# Autodesk Inventor assembly: power
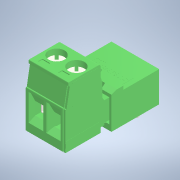
[picture p0: Inventor's stored thumbnail of the model, 180x180]
Saved by Autodesk Inventor 2021 (Build 250183000, 183)
## iProperties
Created: 2023-08-06
Part Number: power
Document SubType Name: Assembly
Designer: michal
Author: michal
## Documents named in this file (3)
- C:\Users\micha\OneDrive\Dokumenty\GitHub\escape_room_hw_v2\Enclosure\Commercial\power.iam
- C:\Users\micha\OneDrive\Dokumenty\GitHub\escape_room_hw_v2\Enclosure\Commercial\139343761-9-1754449\1754449.iam
- C:\Users\micha\OneDrive\Dokumenty\GitHub\escape_room_hw_v2\Enclosure\Commercial\139343763-9-1757475\1757475.iam
## Components (2 placed, 2 different names)
1. 1754449:1 [sub-assembly] — Mate:1, Mate:2, Mate:3
2. 1757475:1 [sub-assembly] — Mate:1, Mate:2, Mate:3
## Relationships (3: Mate 3)
- Mate:1: 1754449:1 ↔ 1757475:1
- Mate:2: 1754449:1 ↔ 1757475:1
- Mate:3: 1754449:1 ↔ 1757475:1
